# Autodesk Inventor assembly: Montagem1
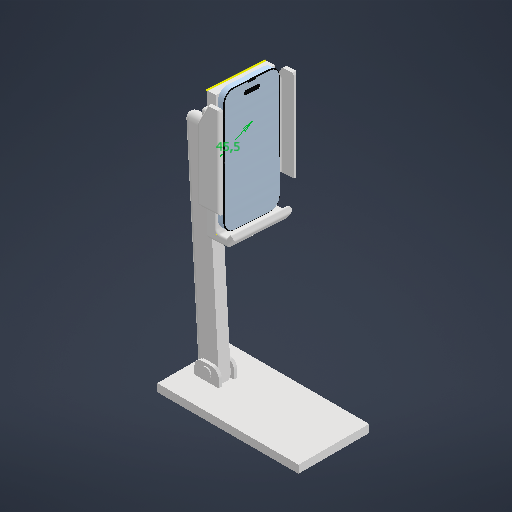
[picture p0: Inventor's stored thumbnail of the model, 512x512]
Saved by Autodesk Inventor 2027 (Build 310192060, 192F)
## iProperties
Created: 2026-10-07
Part Number: Montagem1
Document SubType Name: Assembly
Designer: guisg
Author: guisg
## Documents named in this file (6)
- C:\Users\guisg\Downloads\cp_CAD_Iphone\Montagem1.iam
- C:\Users\guisg\Downloads\suporte.ipt
- C:\Users\guisg\Downloads\cilindro meio.ipt
- C:\Users\guisg\Downloads\cp_CAD_Iphone\Iphone17.ipt
- C:\Users\guisg\Downloads\base.ipt
- C:\Users\guisg\Downloads\braço.ipt
## Components (5 placed, 5 different names)
1. suporte:1 — Inserir:1, Inserir:3, Rígida:1
2. cilindro meio:1 — Inserir:1, Inserir:2, Inserir:4
3. base:1 — Inserir:2, Coincidente:1, Coincidente:2
4. braço:1 — Coincidente:1, Coincidente:2, Inserir:3, Inserir:4
5. Iphone17:1 — Rígida:1
## Relationships (7: Insert 4, Mate 2, WeldJoint 1)
- Inserir:1 (-4 mm): suporte:1 ↔ cilindro meio:1
- Inserir:2 (-4 mm): cilindro meio:1 ↔ base:1
- Coincidente:1 [Mate]: base:1 ↔ braço:1
- Coincidente:2 [Mate]: base:1 ↔ braço:1
- Inserir:3: suporte:1 ↔ braço:1
- Inserir:4 (-6 mm): cilindro meio:1 ↔ braço:1
- Rígida:1 [WeldJoint]: suporte:1 ↔ Iphone17:1
